# Autodesk Inventor assembly: Servo Mechanism
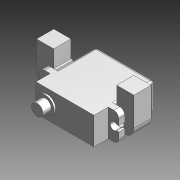
[picture p0: Inventor's stored thumbnail of the model, 180x180]
Saved by Autodesk Inventor 2014 SP1 (Build 180222100, 222)
## iProperties
Created: 2013-12-25
Part Number: Servo Mechanism
Document SubType Name: Assembly
Designer: tom
Author: tom
## Documents named in this file (3)
- C:\Users\tom\Documents\GitHub\Delta_Robots\Delatabot - Small Model\Imported Components\Deltabot - Small Model\Servo Mechanism.iam
- C:\Users\tom\Documents\GitHub\Delta_Robots\Delatabot - Small Model\Imported Components\Deltabot - Small Model\Component2.ipt
- C:\Users\tom\Documents\GitHub\Delta_Robots\Delatabot - Small Model\Imported Components\Deltabot - Small Model\Component12.ipt
## Components (3 placed, 3 different names)
1. Servo
2. Servo Bracket 1
3. Servo Bracket 2
## Relationships (6: Mate 6)
- [Mate] (0.1225 mm): Servo ↔ Servo Bracket 2
- [Mate] (0.1225 mm): Servo ↔ Servo Bracket 1
- [Mate] (0.1225 mm): Servo ↔ Servo Bracket 1
- [Mate] (0.1225 mm): Servo ↔ Servo Bracket 2
- [Mate]: Servo ↔ Servo Bracket 2
- [Mate]: Servo ↔ Servo Bracket 1
